# Autodesk Inventor assembly: Gantry
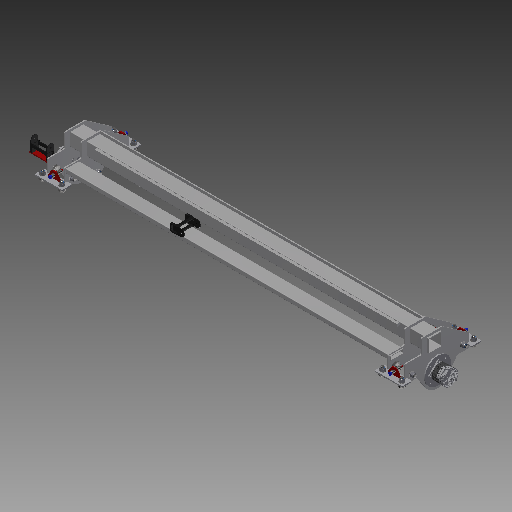
[picture p0: Inventor's stored thumbnail of the model, 512x512]
Saved by Autodesk Inventor 2018.2 (Build 222227000, 227)
## iProperties
Created: 2017-12-18
Part Number: Gantry
Document SubType Name: Assembly
Designer: torba
Author: torba
## Documents named in this file (19)
- C:\Users\torba\OneDrive\Documents\Inventor\Plasma 5x10\Gantry.iam
- C:\Users\torba\OneDrive\Documents\Inventor\Plasma 5x10\3 x 3 TUBE .125 steel\3 x 3 TUBE .125 steel-81.75.ipt
- C:\Users\torba\OneDrive\Documents\Inventor\Plasma 5x10\3 x 3 TUBE .125 steel.ipt
- C:\Users\torba\OneDrive\Documents\Inventor\Plasma 5x10\4x.25 cold rolled steel.ipt
- C:\Users\torba\OneDrive\Documents\Inventor\Plasma 5x10\gantry inner.ipt
- C:\Users\torba\OneDrive\Documents\Inventor\Plasma 5x10\1 x 3 tube .125.ipt
- C:\Users\torba\OneDrive\Documents\Inventor\Plasma 5x10\1 x 3 tube .125\1 x 3 tube .125-74.ipt
- C:\Users\torba\OneDrive\Documents\Inventor\Plasma 5x10\Gantry Outer.ipt
- C:\Users\torba\OneDrive\Documents\Inventor\Plasma 5x10\CPM-341x\CPM-_ _ _ _ - 3411_-LS.ipt
- C:\Users\torba\OneDrive\Documents\Inventor\Plasma 5x10\Gantry Side load assy.iam
- C:\Users\torba\OneDrive\Documents\Inventor\Plasma 5x10\Servo Flange.ipt
- C:\Users\torba\OneDrive\Documents\Inventor\Plasma 5x10\PSC1024 Gear (Simplified).ipt
- C:\Users\torba\OneDrive\Documents\Inventor\Plasma 5x10\Bearing Assembly.iam
- C:\Users\torba\OneDrive\Documents\Inventor\Plasma 5x10\RSHC10XX00 Rack (Simplified)\RSHC10XX00 Rack (Simplified)-68.5.ipt
- C:\Users\torba\OneDrive\Documents\Inventor\Plasma 5x10\RSHC10XX00 Rack (Simplified).ipt
- C:\Users\torba\OneDrive\Documents\Inventor\Plasma 5x10\Drag Chain End.ipt
- C:\Users\torba\OneDrive\Documents\Inventor\Plasma 5x10\Gantry Chain Support.ipt
- C:\Users\torba\OneDrive\Documents\Inventor\Plasma 5x10\Limit Switch.ipt
- C:\Users\torba\OneDrive\Documents\Inventor\Plasma 5x10\Limit Mount.ipt
## Components (41 placed, 15 different names)
1. 3 x 3 TUBE .125 steel-81.75:2 — Mate:1, Flush:1, Flush:2, Mate:2, Mate:3, Mate:6, Mate:7, Flush:4, Flush:5, Mate:76, Mate:77, Mate:81, Mate:132, Mate:138, Flush:20
2. 4x.25 cold rolled steel:1 — Mate:1, Flush:1, Flush:2, Mate:20, Mate:21
3. gantry inner:1 — Mate:3, Mate:6, Mate:20, Mate:111, Mate:112, Mate:113, Mate:125, Mate:127, Mate:128, Flush:25, Mate:157
4. gantry inner:2 — Mate:2, Mate:7, Mate:21, Mate:22, Mate:23, Flush:3, Mate:117, Mate:118, Mate:119, Mate:121, Mate:122, Mate:123, Mate:139, Mate:150, Flush:26, Mate:156
5. 1 x 3 tube .125-74:1 — Mate:22, Mate:23, Flush:3, Mate:149, Flush:22
6. Gantry Outer:1 — Flush:5, Mate:76, Mate:77, Mate:86, Mate:115, Mate:116, Mate:120, Mate:124, Mate:133, Mate:135, Mate:137, Mate:140, Mate:141, Mate:147, Angle:2, Mate:153, Flush:23, Flush:24
7. Gantry Outer:2 — Flush:4, Mate:81, Mate:110, Mate:114, Mate:126, Mate:129, Mate:131, Mate:132, Mate:134, Mate:148, Angle:1
8. PSC1024 Gear (Simplified):1 — Flush:14, Mate:109, Mate:146, Mate:147
9. CPM-_ _ _ _ - 3411_-LS:1 — Mate:83, Mate:85, Mate:87, Flush:14, Mate:109, Angle:2
10. Servo Flange:1 — Mate:83, Mate:85, Mate:86, Mate:87
11. Bearing Assembly:1 [sub-assembly] — Mate:110, Mate:129
12. Bearing Assembly:2 [sub-assembly] — Mate:113, Mate:125
13. Bearing Assembly:3 [sub-assembly] — Mate:111, Mate:128
14. Bearing Assembly:4 [sub-assembly] — Mate:116, Mate:120
15. Bearing Assembly:5 [sub-assembly] — Mate:112, Mate:127
16. Bearing Assembly:6 [sub-assembly] — Mate:117, Mate:122
17. Bearing Assembly:7 [sub-assembly] — Mate:118, Mate:123
18. Bearing Assembly:8 [sub-assembly] — Mate:119, Mate:121
19. Bearing Assembly:9 [sub-assembly] — Mate:114, Mate:126
20. Bearing Assembly:10 [sub-assembly] — Mate:115, Mate:124
21. RSHC10XX00 Rack (Simplified)-68.5:1 — Mate:138, Flush:20, Mate:139
22. Gantry Side load assy:5 [sub-assembly] — Flush:15, Flush:19, Mate:133, Mate:141, Mate:160, Flush:30, Flush:34
23. Gantry Side load assy:6 [sub-assembly] — Flush:16, Flush:17, Flush:18, Mate:134, Flush:33
24. Gantry Side load assy:7 [sub-assembly] — Flush:17, Flush:18, Mate:135, Mate:137, Mate:140, Flush:31
25. Gantry Side load assy:8 [sub-assembly] — Flush:15, Flush:16, Flush:19, Mate:131, Mate:161, Flush:32, Flush:35
26. CPM-_ _ _ _ - 3411_-LS:2 — Angle:1
27. Servo Flange:2 — Mate:148
28. PSC1024 Gear (Simplified):2 — Mate:146
29. Drag Chain End:1 — Mate:149, Flush:22, Mate:150
30. Drag Chain End:2 — Mate:154, Mate:155
31. Gantry Chain Support:1 — Mate:153, Flush:23, Flush:24, Mate:154, Mate:155
32. Limit Switch:1 — Flush:25, Mate:157
33. Limit Switch:2 — Flush:26, Mate:156
34. Limit Mount:1 — Flush:27, Mate:159, Mate:161, Flush:32, Flush:35, Mate:164, Flush:37
35. Limit Mount:2 — Flush:27, Flush:28, Mate:159, Flush:33, Mate:165, Flush:36
36. Limit Mount:3 — Flush:28, Flush:29, Mate:158, Mate:160, Flush:30, Flush:34, Mate:162, Flush:39
37. Limit Mount:4 — Flush:29, Mate:158, Flush:31, Mate:163, Flush:38
38. Limit Switch:3 — Mate:165, Flush:36
39. Limit Switch:4 — Mate:164, Flush:37
40. Limit Switch:5 — Mate:163, Flush:38
41. Limit Switch:6 — Mate:162, Flush:39
## Relationships (102: Mate 69, Flush 31, Angle 2)
- Mate:1: 3 x 3 TUBE .125 steel-81.75:2 ↔ 4x.25 cold rolled steel:1
- Flush:1 (-111.125 mm): 3 x 3 TUBE .125 steel-81.75:2 ↔ 4x.25 cold rolled steel:1
- Flush:2 (-12.7 mm): 3 x 3 TUBE .125 steel-81.75:2 ↔ 4x.25 cold rolled steel:1
- Mate:2: 3 x 3 TUBE .125 steel-81.75:2 ↔ gantry inner:2
- Mate:3: 3 x 3 TUBE .125 steel-81.75:2 ↔ gantry inner:1
- Mate:6: 3 x 3 TUBE .125 steel-81.75:2 ↔ gantry inner:1
- Mate:7: 3 x 3 TUBE .125 steel-81.75:2 ↔ gantry inner:2
- Mate:20: 4x.25 cold rolled steel:1 ↔ gantry inner:1
- Mate:21: 4x.25 cold rolled steel:1 ↔ gantry inner:2
- Mate:22: gantry inner:2 ↔ 1 x 3 tube .125-74:1
- Mate:23: gantry inner:2 ↔ 1 x 3 tube .125-74:1
- Flush:3 (-6.35 mm): gantry inner:2 ↔ 1 x 3 tube .125-74:1
- Flush:4 (9.525 mm): 3 x 3 TUBE .125 steel-81.75:2 ↔ Gantry Outer:2
- Flush:5 (9.525 mm): 3 x 3 TUBE .125 steel-81.75:2 ↔ Gantry Outer:1
- Mate:76: 3 x 3 TUBE .125 steel-81.75:2 ↔ Gantry Outer:1
- Mate:77: 3 x 3 TUBE .125 steel-81.75:2 ↔ Gantry Outer:1
- Mate:81: 3 x 3 TUBE .125 steel-81.75:2 ↔ Gantry Outer:2
- Mate:83: CPM-_ _ _ _ - 3411_-LS:1 ↔ Servo Flange:1
- Mate:85: CPM-_ _ _ _ - 3411_-LS:1 ↔ Servo Flange:1
- Mate:86: Gantry Outer:1 ↔ Servo Flange:1
- Mate:87: CPM-_ _ _ _ - 3411_-LS:1 ↔ Servo Flange:1
- Flush:14: PSC1024 Gear (Simplified):1 ↔ CPM-_ _ _ _ - 3411_-LS:1
- Mate:109: PSC1024 Gear (Simplified):1 ↔ CPM-_ _ _ _ - 3411_-LS:1
- Mate:110: Gantry Outer:2 ↔ Bearing Assembly:1
- Mate:111: gantry inner:1 ↔ Bearing Assembly:3
- Mate:112: gantry inner:1 ↔ Bearing Assembly:5
- Mate:113: gantry inner:1 ↔ Bearing Assembly:2
- Mate:114: Gantry Outer:2 ↔ Bearing Assembly:9
- Mate:115: Gantry Outer:1 ↔ Bearing Assembly:10
- Mate:116: Gantry Outer:1 ↔ Bearing Assembly:4
- Mate:117: gantry inner:2 ↔ Bearing Assembly:6
- Mate:118: gantry inner:2 ↔ Bearing Assembly:7
- Mate:119: gantry inner:2 ↔ Bearing Assembly:8
- Mate:120: Gantry Outer:1 ↔ Bearing Assembly:4
- Mate:121: gantry inner:2 ↔ Bearing Assembly:8
- Mate:122: gantry inner:2 ↔ Bearing Assembly:6
- Mate:123: gantry inner:2 ↔ Bearing Assembly:7
- Mate:124: Gantry Outer:1 ↔ Bearing Assembly:10
- Mate:125: gantry inner:1 ↔ Bearing Assembly:2
- Mate:126: Gantry Outer:2 ↔ Bearing Assembly:9
- Mate:127: gantry inner:1 ↔ Bearing Assembly:5
- Mate:128: gantry inner:1 ↔ Bearing Assembly:3
- Mate:129: Gantry Outer:2 ↔ Bearing Assembly:1
- Flush:15: Gantry Side load assy:5 ↔ Gantry Side load assy:8
- Flush:16: Gantry Side load assy:6 ↔ Gantry Side load assy:8
- Flush:17: Gantry Side load assy:6 ↔ Gantry Side load assy:7
- Flush:18: Gantry Side load assy:6 ↔ Gantry Side load assy:7
- Flush:19: Gantry Side load assy:5 ↔ Gantry Side load assy:8
- Mate:131: Gantry Outer:2 ↔ Gantry Side load assy:8
- Mate:132: 3 x 3 TUBE .125 steel-81.75:2 ↔ Gantry Outer:2
- Mate:133: Gantry Outer:1 ↔ Gantry Side load assy:5
- Mate:134: Gantry Outer:2 ↔ Gantry Side load assy:6
- Mate:135: Gantry Outer:1 ↔ Gantry Side load assy:7
- Mate:137 (-19.0246 mm): Gantry Outer:1 ↔ Gantry Side load assy:7
- Mate:138: 3 x 3 TUBE .125 steel-81.75:2 ↔ RSHC10XX00 Rack (Simplified)-68.5:1
- Flush:20 (3.175 mm): 3 x 3 TUBE .125 steel-81.75:2 ↔ RSHC10XX00 Rack (Simplified)-68.5:1
- Mate:139 (57.15 mm): gantry inner:2 ↔ RSHC10XX00 Rack (Simplified)-68.5:1
- Mate:140: Gantry Outer:1 ↔ Gantry Side load assy:7
- Mate:141: Gantry Outer:1 ↔ Gantry Side load assy:5
- [Mate]: CPM-_ _ _ _ - 3411_-LS:2 ↔ Servo Flange:2
- [Mate]: CPM-_ _ _ _ - 3411_-LS:2 ↔ Servo Flange:2
- [Mate]: CPM-_ _ _ _ - 3411_-LS:2 ↔ Servo Flange:2
- [Flush]: CPM-_ _ _ _ - 3411_-LS:2 ↔ PSC1024 Gear (Simplified):2
- [Mate]: CPM-_ _ _ _ - 3411_-LS:2 ↔ PSC1024 Gear (Simplified):2
- Mate:146: PSC1024 Gear (Simplified):1 ↔ PSC1024 Gear (Simplified):2
- Mate:147: Gantry Outer:1 ↔ PSC1024 Gear (Simplified):1
- Mate:148: Gantry Outer:2 ↔ Servo Flange:2
- Angle:1 (225 deg): Gantry Outer:2 ↔ CPM-_ _ _ _ - 3411_-LS:2
- Angle:2 (-45 deg): Gantry Outer:1 ↔ CPM-_ _ _ _ - 3411_-LS:1
- Mate:149: 1 x 3 tube .125-74:1 ↔ Drag Chain End:1
- Flush:22 (-11.8999 mm): 1 x 3 tube .125-74:1 ↔ Drag Chain End:1
- Mate:150 (609.6 mm): gantry inner:2 ↔ Drag Chain End:1
- Mate:153: Gantry Outer:1 ↔ Gantry Chain Support:1
- Flush:23 (-25.4 mm): Gantry Outer:1 ↔ Gantry Chain Support:1
- Flush:24 (-6.35 mm): Gantry Outer:1 ↔ Gantry Chain Support:1
- Mate:154: Drag Chain End:2 ↔ Gantry Chain Support:1
- Mate:155: Drag Chain End:2 ↔ Gantry Chain Support:1
- Flush:25 (25.4 mm): gantry inner:1 ↔ Limit Switch:1
- Flush:26 (-25.4 mm): gantry inner:2 ↔ Limit Switch:2
- Mate:156: gantry inner:2 ↔ Limit Switch:2
- Mate:157: gantry inner:1 ↔ Limit Switch:1
- Flush:27: Limit Mount:1 ↔ Limit Mount:2
- Flush:28: Limit Mount:2 ↔ Limit Mount:3
- Flush:29: Limit Mount:3 ↔ Limit Mount:4
- Mate:158: Limit Mount:3 ↔ Limit Mount:4
- Mate:159: Limit Mount:1 ↔ Limit Mount:2
- Mate:160: Gantry Side load assy:5 ↔ Limit Mount:3
- Mate:161: Gantry Side load assy:8 ↔ Limit Mount:1
- Flush:30 (31.75 mm): Gantry Side load assy:5 ↔ Limit Mount:3
- Flush:31 (31.75 mm): Gantry Side load assy:7 ↔ Limit Mount:4
- Flush:32 (31.75 mm): Gantry Side load assy:8 ↔ Limit Mount:1
- Flush:33 (31.75 mm): Gantry Side load assy:6 ↔ Limit Mount:2
- Flush:34 (-45.466 mm): Gantry Side load assy:5 ↔ Limit Mount:3
- Flush:35 (45.466 mm): Gantry Side load assy:8 ↔ Limit Mount:1
- Mate:162: Limit Mount:3 ↔ Limit Switch:6
- Mate:163: Limit Mount:4 ↔ Limit Switch:5
- Mate:164: Limit Mount:1 ↔ Limit Switch:4
- Mate:165: Limit Mount:2 ↔ Limit Switch:3
- Flush:36 (-25.4 mm): Limit Mount:2 ↔ Limit Switch:3
- Flush:37 (-25.4 mm): Limit Mount:1 ↔ Limit Switch:4
- Flush:38 (-25.4 mm): Limit Mount:4 ↔ Limit Switch:5
- Flush:39 (-25.4 mm): Limit Mount:3 ↔ Limit Switch:6
## Named parameters: d182_d141 = 0 mm, d183_d142 = 0 mm, d184_d115 = 0 mm, d185_d117 = 0 mm, d186_d113 = 0 mm
